# Autodesk Inventor assembly: 5SS_Platform
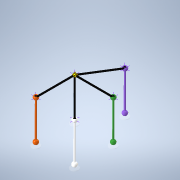
[picture p0: Inventor's stored thumbnail of the model, 180x180]
Saved by Autodesk Inventor 2020.1 (Build 241239000, 239)
## iProperties
Created: 2019-10-24
Part Number: 5SS_Platform
Document SubType Name: Assembly
Designer: sshel
Author: sshel
## Documents named in this file (10)
- D:\Desktop 2019\MS, Phd\Sem8- 2019 Spring (RA, 3research)\Spatial approach- Spherical and Planar synthesis\CAD\5SS Platform (5 redundant dof)\5SS_Platform.iam
- D:\Desktop 2019\MS, Phd\Sem8- 2019 Spring (RA, 3research)\Spatial approach- Spherical and Planar synthesis\CAD\5SS Platform (5 redundant dof)\Components\FP.ipt
- D:\Desktop 2019\MS, Phd\Sem8- 2019 Spring (RA, 3research)\Spatial approach- Spherical and Planar synthesis\CAD\Components\SS_Dyad.ipt
- D:\Desktop 2019\MS, Phd\Sem8- 2019 Spring (RA, 3research)\Spatial approach- Spherical and Planar synthesis\CAD\5SS Platform (5 redundant dof)\Components\SS_Dyad\SS_Dyad-01.ipt
- D:\Desktop 2019\MS, Phd\Sem8- 2019 Spring (RA, 3research)\Spatial approach- Spherical and Planar synthesis\CAD\5SS Platform (5 redundant dof)\Components\SS_Dyad\SS_Dyad-02.ipt
- D:\Desktop 2019\MS, Phd\Sem8- 2019 Spring (RA, 3research)\Spatial approach- Spherical and Planar synthesis\CAD\5SS Platform (5 redundant dof)\Components\SS_Dyad\SS_Dyad-03.ipt
- D:\Desktop 2019\MS, Phd\Sem8- 2019 Spring (RA, 3research)\Spatial approach- Spherical and Planar synthesis\CAD\5SS Platform (5 redundant dof)\Components\SS_Dyad\SS_Dyad-04.ipt
- D:\Desktop 2019\MS, Phd\Sem8- 2019 Spring (RA, 3research)\Spatial approach- Spherical and Planar synthesis\CAD\5SS Platform (5 redundant dof)\Components\SS_Dyad\SS_Dyad-05.ipt
- D:\Desktop 2019\MS, Phd\Sem8- 2019 Spring (RA, 3research)\Spatial approach- Spherical and Planar synthesis\CAD\5SS Platform (5 redundant dof)\Components\Coupler.ipt
- D:\Desktop 2019\MS, Phd\Sem8- 2019 Spring (RA, 3research)\Spatial approach- Spherical and Planar synthesis\CAD\5SS Platform (5 redundant dof)\Linked Parameters.xlsx
## Components (11 placed, 7 different names)
1. FP:1 — Flush:3, Ball:1
2. FP:2 — Flush:6, Ball:2
3. FP:3 — Flush:9, Ball:3
4. FP:4 — Flush:12, Ball:4
5. FP:5 — Flush:15, Ball:5
6. SS_Dyad-01:1 — Ball:1, Ball:6
7. SS_Dyad-02:2 — Ball:2, Ball:7
8. SS_Dyad-03:3 — Ball:3, Ball:8
9. SS_Dyad-04:4 — Ball:4, Ball:9
10. SS_Dyad-05:5 — Ball:5, Ball:10
11. Coupler:1 — Ball:6, Ball:7, Ball:8, Ball:9, Ball:10
## Relationships (25: Flush 15, BallJoint 10)
- [Flush]: FP:1
- [Flush]: FP:1
- Flush:3: FP:1
- [Flush]: FP:2
- [Flush]: FP:2
- Flush:6: FP:2
- [Flush]: FP:3
- [Flush]: FP:3
- Flush:9: FP:3
- [Flush]: FP:4
- [Flush]: FP:4
- Flush:12: FP:4
- [Flush]: FP:5
- [Flush]: FP:5
- Flush:15: FP:5
- Ball:1: FP:1 ↔ SS_Dyad-01:1
- Ball:2: FP:2 ↔ SS_Dyad-02:2
- Ball:3: FP:3 ↔ SS_Dyad-03:3
- Ball:4: FP:4 ↔ SS_Dyad-04:4
- Ball:5: FP:5 ↔ SS_Dyad-05:5
- Ball:6: SS_Dyad-01:1 ↔ Coupler:1
- Ball:7: SS_Dyad-02:2 ↔ Coupler:1
- Ball:8: SS_Dyad-03:3 ↔ Coupler:1
- Ball:9: SS_Dyad-04:4 ↔ Coupler:1
- Ball:10: SS_Dyad-05:5 ↔ Coupler:1
## Named parameters: dyad1_Fx = 0 mm, dyad1_Fy = 0 mm, dyad1_Fz = 0 mm, dyad5_Fy = 500 mm, dyad5_Fx = 1800 mm, dyad5_Fz = 0 mm, dyad4_Fz = 0 mm, dyad4_Fy = 1000 mm, dyad4_Fx = 1000 mm, dyad3_Fz = 0 mm, dyad3_Fx = 0 mm, dyad2_Fz = 0 mm, dyad3_Fy = 1000 mm, dyad2_Fx = 1000 mm, dyad2_Fy = 0 mm, L1 = 1000 mm, L2 = 1000 mm, L3 = 1000 mm, L4 = 1000 mm, L5 = 1000 mm, dyad1_mx = 0 mm, dyad1_my = 0 mm, dyad1_mz = -1000 mm, dyad2_mx = 1000 mm, dyad2_my = 0 mm, dyad2_mz = -1000 mm, dyad3_mx = 0 mm, dyad3_my = 1000 mm, dyad3_mz = -1000 mm, dyad4_mx = 1000 mm, dyad4_my = 1000 mm, dyad4_mz = -1000 mm, dyad5_mx = 1800 mm, dyad5_my = 500 mm, dyad5_mz = -1000 mm
